# Autodesk Inventor assembly: Assembly1final
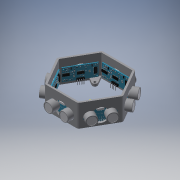
[picture p0: Inventor's stored thumbnail of the model, 180x180]
Saved by Autodesk Inventor 2018 (Build 220112000, 112)
## iProperties
Created: 2017-05-13
Part Number: Assembly1final
Document SubType Name: Assembly
Designer: Vidal Villegas
Author: Vidal Villegas
## Documents named in this file (10)
- C:\Users\Vidal Villegas\Desktop\mp\Assembly1final.iam
- C:\Users\Vidal Villegas\Desktop\mp\megapr.ipt
- C:\Users\Vidal Villegas\Desktop\mp\tornillo.ipt
- C:\Users\Vidal Villegas\Desktop\mp\radar.ipt
- C:\Users\Vidal Villegas\Desktop\mp\portabateria.ipt
- C:\Users\Vidal Villegas\Desktop\mp\lipo.bateria.ipt
- C:\Users\Vidal Villegas\Desktop\mp\User-Library-HC-SR04.iam
- C:\Users\Vidal Villegas\Desktop\mp\tapa.ipt
- C:\Users\Vidal Villegas\Desktop\mp\portaswitch.ipt
- C:\Users\Vidal Villegas\Desktop\mp\switch\41874.iam
## Components (21 placed, 9 different names)
1. megapr:1 — Mate:1, Mate:2, Mate:3, Mate:4, Flush:1, Flush:2, Flush:3, Flush:4, Mate:15
2. tornillo:1 — Mate:1, Flush:4, Mate:6, Mate:19, Mate:28
3. tornillo:2 — Mate:2, Flush:1, Mate:8, Mate:18, Mate:27
4. tornillo:3 — Mate:3, Flush:2, Mate:9, Mate:11, Mate:20, Mate:24
5. tornillo:4 — Mate:4, Flush:3, Mate:7, Mate:10, Mate:21, Mate:25
6. portabateria:1 — Mate:6, Mate:7, Mate:12, Flush:5
7. portabateria:2 — Mate:8, Mate:9, Mate:13, Mate:16, Mate:17
8. radar:1 — Mate:10, Mate:11, Insert:1, Mate:14, Insert:2, Insert:3, Insert:4, Insert:5, Insert:6, Insert:7, Insert:8, Insert:9, Insert:10, Insert:11, Mate:26
9. lipo.bateria:1 — Mate:12, Flush:5, Mate:13, Mate:15, Mate:16, Flush:6, Flush:7
10. lipo.bateria:2 — Mate:17, Flush:6, Flush:7, Mate:22, Mate:23
11. User-Library-HC-SR04:1 [sub-assembly] — Insert:1, Mate:14
12. User-Library-HC-SR04:2 [sub-assembly] — Insert:4, Insert:9
13. User-Library-HC-SR04:3 [sub-assembly] — Insert:2, Insert:3
14. User-Library-HC-SR04:4 [sub-assembly] — Insert:5, Insert:6
15. User-Library-HC-SR04:5 [sub-assembly] — Insert:7, Insert:8
16. User-Library-HC-SR04:6 [sub-assembly] — Insert:10, Insert:11
17. portabateria:3 — Mate:19, Mate:21, Mate:23
18. portabateria:4 — Mate:18, Mate:20, Mate:22
19. tapa:1 — Mate:24, Mate:25, Mate:26
20. portaswitch:1 — Mate:27, Mate:28, Insert:12, Angle:1
21. 41874:1 [sub-assembly] — Insert:12, Angle:1
## Relationships (47: Mate 27, Insert 12, Flush 7, Angle 1)
- Mate:1: megapr:1 ↔ tornillo:1
- Mate:2: megapr:1 ↔ tornillo:2
- Mate:3: megapr:1 ↔ tornillo:3
- Mate:4: megapr:1 ↔ tornillo:4
- Flush:1: megapr:1 ↔ tornillo:2
- Flush:2: megapr:1 ↔ tornillo:3
- Flush:3: megapr:1 ↔ tornillo:4
- Flush:4: megapr:1 ↔ tornillo:1
- Mate:6: tornillo:1 ↔ portabateria:1
- Mate:7: tornillo:4 ↔ portabateria:1
- Mate:8: tornillo:2 ↔ portabateria:2
- Mate:9: tornillo:3 ↔ portabateria:2
- Mate:10: tornillo:4 ↔ radar:1
- Mate:11: tornillo:3 ↔ radar:1
- Mate:12: portabateria:1 ↔ lipo.bateria:1
- Flush:5 (-4 mm): portabateria:1 ↔ lipo.bateria:1
- Mate:13: portabateria:2 ↔ lipo.bateria:1
- Insert:1: radar:1 ↔ User-Library-HC-SR04:1
- Mate:14: radar:1 ↔ User-Library-HC-SR04:1
- Insert:2: radar:1 ↔ User-Library-HC-SR04:3
- Insert:3: radar:1 ↔ User-Library-HC-SR04:3
- Insert:4: radar:1 ↔ User-Library-HC-SR04:2
- Insert:5: radar:1 ↔ User-Library-HC-SR04:4
- Insert:6: radar:1 ↔ User-Library-HC-SR04:4
- Insert:7: radar:1 ↔ User-Library-HC-SR04:5
- Insert:8: radar:1 ↔ User-Library-HC-SR04:5
- Insert:9: radar:1 ↔ User-Library-HC-SR04:2
- Insert:10: radar:1 ↔ User-Library-HC-SR04:6
- Insert:11: radar:1 ↔ User-Library-HC-SR04:6
- Mate:15: megapr:1 ↔ lipo.bateria:1
- Mate:16 (5 mm): portabateria:2 ↔ lipo.bateria:1
- Mate:17: portabateria:2 ↔ lipo.bateria:2
- Flush:6: lipo.bateria:1 ↔ lipo.bateria:2
- Flush:7: lipo.bateria:1 ↔ lipo.bateria:2
- Mate:18: tornillo:2 ↔ portabateria:4
- Mate:19: tornillo:1 ↔ portabateria:3
- Mate:20: tornillo:3 ↔ portabateria:4
- Mate:21: tornillo:4 ↔ portabateria:3
- Mate:22: lipo.bateria:2 ↔ portabateria:4
- Mate:23: lipo.bateria:2 ↔ portabateria:3
- Mate:24: tornillo:3 ↔ tapa:1
- Mate:25: tornillo:4 ↔ tapa:1
- Mate:26: radar:1 ↔ tapa:1
- Mate:27: tornillo:2 ↔ portaswitch:1
- Mate:28: tornillo:1 ↔ portaswitch:1
- Insert:12: portaswitch:1 ↔ 41874:1
- Angle:1 (0 deg): portaswitch:1 ↔ 41874:1
